# Autodesk Inventor assembly: Tube Holder assembly
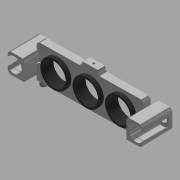
[picture p0: Inventor's stored thumbnail of the model, 180x180]
Saved by Autodesk Inventor 2017 (Build 210142000, 142)
## iProperties
Created: 2017-02-22
Part Number: Tube Holder assembly
Document SubType Name: Assembly
Designer: qupec
Author: qupec
## Documents named in this file (5)
- C:\Users\qupec\Desktop\UMD Near Space\STAR\CAD\Mechanical\Tube Holder assembly.iam
- C:\Users\qupec\Desktop\UMD Near Space\STAR\CAD\Mechanical\Tube Holder Halve 2.ipt
- C:\Users\qupec\Desktop\UMD Near Space\STAR\CAD\Mechanical\Tube Holder Halve.ipt
- C:\Users\qupec\Desktop\UMD Near Space\STAR\CAD\Mechanical\Tube grip.ipt
- C:\Users\qupec\Documents\Inventor\Content Center Files\R2017\en-US\U UNC 2603(1)\Unbrako - 5 x 1 - 40 - 1 - Unbrako.ipt
## Components (7 placed, 4 different names)
1. Tube Holder Halve 2:1 — Mate:1, Mate:2, Flush:1, Mate:3, Mate:4, Mate:5, Flush:2, Flush:3, Flush:4
2. Tube Holder Halve:1 — Mate:1, Mate:2, Flush:1, Insert:1, Insert:2
3. Tube grip:1 — Mate:4, Flush:3
4. Tube grip:2 — Mate:3, Flush:4
5. Tube grip:3 — Mate:5, Flush:2
6. Unbrako UNC Hex Socket Cap - Inch 5 x 1:1 — Insert:1
7. Unbrako UNC Hex Socket Cap - Inch 5 x 1:2 — Insert:2
## Relationships (11: Mate 5, Flush 4, Insert 2)
- Mate:1: Tube Holder Halve 2:1 ↔ Tube Holder Halve:1
- Mate:2: Tube Holder Halve 2:1 ↔ Tube Holder Halve:1
- Flush:1: Tube Holder Halve 2:1 ↔ Tube Holder Halve:1
- Mate:3: Tube Holder Halve 2:1 ↔ Tube grip:2
- Mate:4: Tube Holder Halve 2:1 ↔ Tube grip:1
- Mate:5: Tube Holder Halve 2:1 ↔ Tube grip:3
- Flush:2: Tube Holder Halve 2:1 ↔ Tube grip:3
- Flush:3: Tube Holder Halve 2:1 ↔ Tube grip:1
- Flush:4: Tube Holder Halve 2:1 ↔ Tube grip:2
- Insert:1: Tube Holder Halve:1 ↔ Unbrako UNC Hex Socket Cap - Inch 5 x 1:1
- Insert:2: Tube Holder Halve:1 ↔ Unbrako UNC Hex Socket Cap - Inch 5 x 1:2
